# Autodesk Inventor assembly: BOX_PART
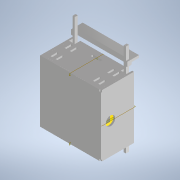
[picture p0: Inventor's stored thumbnail of the model, 180x180]
Saved by Autodesk Inventor 2020 (Build 240168000, 168)
## iProperties
Created: 2019-12-17
Part Number: BOX_PART
Document SubType Name: Assembly
Designer: fabfarm
Author: fabfarm
## Documents named in this file (6)
- D:\fablab\save\BOX_PART.iam
- D:\fablab\save\Side_one.ipt
- D:\fablab\save\Side_two.ipt
- D:\fablab\save\TableSaw_Bench3.ipt
- D:\fablab\save\bottom-case.ipt
- D:\fablab\save\open_case.ipt
## Components (6 placed, 5 different names)
1. Side_one:1 — Mate:9, Mate:12, Flush:4, Mate:13, Flush:5, Symmetry:1
2. Side_two:1 — Mate:10, Mate:12, Flush:4, Mate:13, Flush:7, Symmetry:2
3. TableSaw_Bench3:1 — Flush:6, Flush:9
4. Side_one:2 — Mate:14, Flush:6, Flush:7, Flush:8, Mate:15, Flush:10, Symmetry:1
5. bottom-case:1 — Mate:9, Mate:10, Flush:5, Mate:14, Flush:8
6. open_case:1 — Flush:9, Mate:15, Flush:10, Symmetry:2
## Relationships (15: Flush 7, Mate 6, Symmetry 2)
- Mate:9: Side_one:1 ↔ bottom-case:1
- Mate:10: Side_two:1 ↔ bottom-case:1
- Mate:12: Side_one:1 ↔ Side_two:1
- Flush:4: Side_one:1 ↔ Side_two:1
- Mate:13: Side_one:1 ↔ Side_two:1
- Flush:5: Side_one:1 ↔ bottom-case:1
- Mate:14: Side_one:2 ↔ bottom-case:1
- Flush:6: TableSaw_Bench3:1 ↔ Side_one:2
- Flush:7: Side_two:1 ↔ Side_one:2
- Flush:8: Side_one:2 ↔ bottom-case:1
- Flush:9: TableSaw_Bench3:1 ↔ open_case:1
- Mate:15: Side_one:2 ↔ open_case:1
- Flush:10: Side_one:2 ↔ open_case:1
- Symmetry:1: Side_one:1 ↔ Side_one:2
- Symmetry:2: Side_two:1 ↔ open_case:1
